# Autodesk Inventor assembly: CoinFeeder
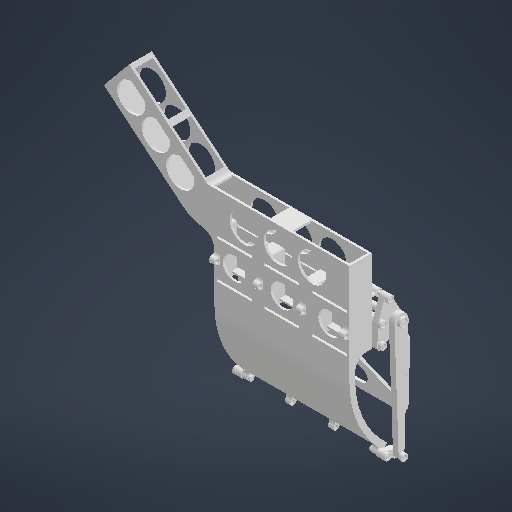
[picture p0: Inventor's stored thumbnail of the model, 512x512]
Saved by Autodesk Inventor 2026.3 (Build 303398000, 398)
## iProperties
Created: 2026-05-05
Part Number: CoinFeeder
Document SubType Name: Assembly
Designer: frede
Author: frede
## Documents named in this file (12)
- E:\Git\AppliedAutomationProject\feeder\trayFeeder\CoinFeeder.iam
- E:\Git\AppliedAutomationProject\feeder\trayFeeder\CoinFeeder.ipt
- E:\Git\AppliedAutomationProject\feeder\trayFeeder\CoinLock.ipt
- E:\Git\AppliedAutomationProject\feeder\trayFeeder\CoinLockOpener.ipt
- E:\Git\AppliedAutomationProject\feeder\trayFeeder\mellemStykke.ipt
- E:\Git\AppliedAutomationProject\feeder\trayFeeder\CoinLockUdløser.ipt
- E:\Git\AppliedAutomationProject\feeder\trayFeeder\step\CoinFeederØ3Rod.ipt
- E:\Git\AppliedAutomationProject\feeder\trayFeeder\Ø(6-3.5)x3.ipt
- E:\Git\AppliedAutomationProject\feeder\trayFeeder\Ø5x145.ipt
- E:\Git\AppliedAutomationProject\feeder\trayFeeder\step\Ø(8-5)x3.ipt
- E:\Git\AppliedAutomationProject\feeder\trayFeeder\Ø3Split.ipt
- E:\Git\AppliedAutomationProject\feeder\trayFeeder\bracing.ipt
## Components (36 placed, 11 different names)
1. CoinFeeder:1 — Mate:1, Mate:2, Mate:3, Mate:4, Mate:5, Mate:6, Mate:7, Mate:8, Mate:9, Mate:10, Mate:11, Mate:12, Flush:1, Mate:13, Mate:16, Mate:17, Mate:18, Mate:19, Mate:20, Mate:21, Flush:2, Mate:32, Mate:33, Mate:34, Mate:63, Mate:64, Mate:65, Mate:66
2. CoinLock:1 — Mate:3, Mate:10, Mate:29, Mate:30
3. CoinLock:2 — Mate:4, Mate:9, Mate:28, Mate:31
4. CoinLock:3 — Mate:6, Mate:7, Mate:14, Mate:22, Mate:41
5. CoinLock:4 — Mate:1, Mate:12, Mate:15, Mate:23, Mate:43
6. CoinLock:5 — Mate:2, Mate:11, Mate:25, Mate:26
7. CoinLock:6 — Mate:5, Mate:8, Mate:24, Mate:27
8. CoinLockOpener:1 — Flush:1, Mate:13, Mate:14, Mate:15, Mate:38, Mate:39, Mate:42, Mate:50, Mate:51, Mate:52
9. CoinLockOpener:2 — Mate:16, Mate:17, Mate:22, Mate:23, Mate:24, Mate:25
10. CoinLockOpener:3 — Mate:18, Mate:19, Mate:26, Mate:27, Mate:28, Mate:29
11. CoinLockOpener:4 — Mate:20, Mate:21, Mate:30, Mate:31, Mate:35, Mate:36
12. mellemStykke:1 — Flush:2, Mate:32, Mate:37, Mate:59, Mate:60
13. mellemStykke:2 — Mate:33, Mate:34, Mate:40, Mate:58
14. CoinLockUdløser:1 — Mate:38, Mate:39, Mate:40, Mate:53, Mate:56, Mate:57, Flush:16, Flush:17
15. CoinLockUdløser:2 — Mate:35, Mate:36, Mate:37
16. CoinFeederØ3Rod:1 — Mate:42, Mate:45, Flush:4, Mate:48, Flush:7
17. CoinFeederØ3Rod:2 — Mate:41, Mate:44, Flush:3, Mate:47, Flush:8
18. CoinFeederØ3Rod:3 — Mate:43, Mate:46, Flush:5, Mate:49, Flush:6
19. Ø(6-3.5)x3:1 — Mate:44, Flush:3, Mate:50
20. Ø(6-3.5)x3:2 — Mate:45, Flush:4, Mate:51
21. Ø(6-3.5)x3:3 — Mate:46, Flush:5, Mate:52
22. Ø(6-3.5)x3:4 — Mate:47, Flush:8
23. Ø(6-3.5)x3:5 — Mate:48, Flush:7
24. Ø(6-3.5)x3:6 — Mate:49, Flush:6
25. Ø5x145:1 — Mate:53, Mate:54, Flush:9, Mate:55, Flush:15
26. Ø(8-5)x3:1 — Mate:54, Flush:9, Mate:56
27. Ø(8-5)x3:2 — Mate:55, Flush:15
28. Ø3Split:1 — Mate:57, Mate:58, Mate:61, Flush:11
29. Ø3Split:2 — Mate:59, Mate:60, Mate:62, Flush:12
30. Ø(6-3.5)x3:7 — Mate:61, Flush:11
31. Ø(6-3.5)x3:8 — Mate:62, Flush:12
32. Ø3Split:3 — Mate:64, Mate:66, Mate:68, Flush:13
33. Ø3Split:4 — Mate:63, Mate:65, Mate:67, Flush:14
34. Ø(6-3.5)x3:9 — Mate:67, Flush:14
35. Ø(6-3.5)x3:10 — Mate:68, Flush:13
36. bracing:1 — Flush:16, Flush:17
## Relationships (84: Mate 68, Flush 16)
- Mate:1 (0.5 mm): CoinFeeder:1 ↔ CoinLock:4
- Mate:2 (0.5 mm): CoinFeeder:1 ↔ CoinLock:5
- Mate:3 (0.5 mm): CoinFeeder:1 ↔ CoinLock:1
- Mate:4 (0.5 mm): CoinFeeder:1 ↔ CoinLock:2
- Mate:5 (0.5 mm): CoinFeeder:1 ↔ CoinLock:6
- Mate:6 (0.5 mm): CoinFeeder:1 ↔ CoinLock:3
- Mate:7 (0.125 mm): CoinFeeder:1 ↔ CoinLock:3
- Mate:8 (0.125 mm): CoinFeeder:1 ↔ CoinLock:6
- Mate:9 (0.125 mm): CoinFeeder:1 ↔ CoinLock:2
- Mate:10 (0.125 mm): CoinFeeder:1 ↔ CoinLock:1
- Mate:11 (0.125 mm): CoinFeeder:1 ↔ CoinLock:5
- Mate:12 (0.125 mm): CoinFeeder:1 ↔ CoinLock:4
- Flush:1: CoinFeeder:1 ↔ CoinLockOpener:1
- Mate:13: CoinFeeder:1 ↔ CoinLockOpener:1
- Mate:14 (1.75 mm): CoinLock:3 ↔ CoinLockOpener:1
- Mate:15 (1.75 mm): CoinLock:4 ↔ CoinLockOpener:1
- Mate:16: CoinFeeder:1 ↔ CoinLockOpener:2
- Mate:17: CoinFeeder:1 ↔ CoinLockOpener:2
- Mate:18: CoinFeeder:1 ↔ CoinLockOpener:3
- Mate:19: CoinFeeder:1 ↔ CoinLockOpener:3
- Mate:20: CoinFeeder:1 ↔ CoinLockOpener:4
- Mate:21: CoinFeeder:1 ↔ CoinLockOpener:4
- Mate:22 (1.75 mm): CoinLock:3 ↔ CoinLockOpener:2
- Mate:23 (1.75 mm): CoinLock:4 ↔ CoinLockOpener:2
- Mate:24 (1.75 mm): CoinLock:6 ↔ CoinLockOpener:2
- Mate:25 (1.75 mm): CoinLock:5 ↔ CoinLockOpener:2
- Mate:26 (1.75 mm): CoinLock:5 ↔ CoinLockOpener:3
- Mate:27 (1.75 mm): CoinLock:6 ↔ CoinLockOpener:3
- Mate:28 (1.75 mm): CoinLock:2 ↔ CoinLockOpener:3
- Mate:29 (1.75 mm): CoinLock:1 ↔ CoinLockOpener:3
- Mate:30 (1.75 mm): CoinLock:1 ↔ CoinLockOpener:4
- Mate:31 (1.75 mm): CoinLock:2 ↔ CoinLockOpener:4
- Flush:2: CoinFeeder:1 ↔ mellemStykke:1
- Mate:32: CoinFeeder:1 ↔ mellemStykke:1
- Mate:33: CoinFeeder:1 ↔ mellemStykke:2
- Mate:34: CoinFeeder:1 ↔ mellemStykke:2
- Mate:35: CoinLockOpener:4 ↔ CoinLockUdløser:2
- Mate:36: CoinLockOpener:4 ↔ CoinLockUdløser:2
- Mate:37: mellemStykke:1 ↔ CoinLockUdløser:2
- Mate:38: CoinLockOpener:1 ↔ CoinLockUdløser:1
- Mate:39: CoinLockOpener:1 ↔ CoinLockUdløser:1
- Mate:40: mellemStykke:2 ↔ CoinLockUdløser:1
- Mate:41: CoinLock:3 ↔ CoinFeederØ3Rod:2
- Mate:42: CoinLockOpener:1 ↔ CoinFeederØ3Rod:1
- Mate:43: CoinLock:4 ↔ CoinFeederØ3Rod:3
- Mate:44: CoinFeederØ3Rod:2 ↔ Ø(6-3.5)x3:1
- Mate:45: CoinFeederØ3Rod:1 ↔ Ø(6-3.5)x3:2
- Mate:46: CoinFeederØ3Rod:3 ↔ Ø(6-3.5)x3:3
- Flush:3: CoinFeederØ3Rod:2 ↔ Ø(6-3.5)x3:1
- Flush:4: CoinFeederØ3Rod:1 ↔ Ø(6-3.5)x3:2
- Flush:5: CoinFeederØ3Rod:3 ↔ Ø(6-3.5)x3:3
- Mate:47: CoinFeederØ3Rod:2 ↔ Ø(6-3.5)x3:4
- Mate:48: CoinFeederØ3Rod:1 ↔ Ø(6-3.5)x3:5
- Mate:49: CoinFeederØ3Rod:3 ↔ Ø(6-3.5)x3:6
- Flush:6: CoinFeederØ3Rod:3 ↔ Ø(6-3.5)x3:6
- Flush:7: CoinFeederØ3Rod:1 ↔ Ø(6-3.5)x3:5
- Flush:8: CoinFeederØ3Rod:2 ↔ Ø(6-3.5)x3:4
- Mate:50: CoinLockOpener:1 ↔ Ø(6-3.5)x3:1
- Mate:51: CoinLockOpener:1 ↔ Ø(6-3.5)x3:2
- Mate:52: CoinLockOpener:1 ↔ Ø(6-3.5)x3:3
- Mate:53: CoinLockUdløser:1 ↔ Ø5x145:1
- Mate:54: Ø5x145:1 ↔ Ø(8-5)x3:1
- Flush:9: Ø5x145:1 ↔ Ø(8-5)x3:1
- Mate:55: Ø5x145:1 ↔ Ø(8-5)x3:2
- Mate:56: CoinLockUdløser:1 ↔ Ø(8-5)x3:1
- Mate:57: CoinLockUdløser:1 ↔ Ø3Split:1
- Mate:58: mellemStykke:2 ↔ Ø3Split:1
- Mate:59: mellemStykke:1 ↔ Ø3Split:2
- Mate:60: mellemStykke:1 ↔ Ø3Split:2
- Mate:61: Ø3Split:1 ↔ Ø(6-3.5)x3:7
- Mate:62: Ø3Split:2 ↔ Ø(6-3.5)x3:8
- Flush:11: Ø3Split:1 ↔ Ø(6-3.5)x3:7
- Flush:12: Ø3Split:2 ↔ Ø(6-3.5)x3:8
- Mate:63: CoinFeeder:1 ↔ Ø3Split:4
- Mate:64: CoinFeeder:1 ↔ Ø3Split:3
- Mate:65: CoinFeeder:1 ↔ Ø3Split:4
- Mate:66: CoinFeeder:1 ↔ Ø3Split:3
- Mate:67: Ø3Split:4 ↔ Ø(6-3.5)x3:9
- Mate:68: Ø3Split:3 ↔ Ø(6-3.5)x3:10
- Flush:13: Ø3Split:3 ↔ Ø(6-3.5)x3:10
- Flush:14: Ø3Split:4 ↔ Ø(6-3.5)x3:9
- Flush:15: Ø5x145:1 ↔ Ø(8-5)x3:2
- Flush:16: CoinLockUdløser:1 ↔ bracing:1
- Flush:17: CoinLockUdløser:1 ↔ bracing:1
